# Autodesk Inventor assembly: puertas
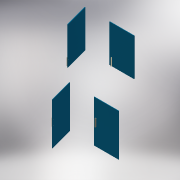
[picture p0: Inventor's stored thumbnail of the model, 180x180]
Saved by Autodesk Inventor 2016 (Build 200138000, 138)
## iProperties
Created: 2015-11-25
Part Number: puertas
Document SubType Name: Assembly
Designer: Daniela
Author: Daniela
## Documents named in this file (4)
- C:\Users\Sebastian\Desktop\sebas\trabajos\COCINA FINAAAAAAAAAAAL\COCINA FINAAAAAAAAAAAL\Cocina\Cocina\puertas.iam
- C:\Users\Sebastian\Desktop\sebas\trabajos\COCINA FINAAAAAAAAAAAL\COCINA FINAAAAAAAAAAAL\Cocina\Cocina\manija.ipt
- C:\Users\Sebastian\Desktop\sebas\trabajos\COCINA FINAAAAAAAAAAAL\COCINA FINAAAAAAAAAAAL\Cocina\Cocina\puerta_inf.ipt
- C:\Users\Sebastian\Desktop\sebas\trabajos\COCINA FINAAAAAAAAAAAL\COCINA FINAAAAAAAAAAAL\Cocina\Cocina\puerta_sup.ipt
## Components (6 placed, 3 different names)
1. puerta_inf:1 — Coincidencia:1, Coincidencia:2, Coincidencia:3, Coincidencia:4, Coincidencia:5, Coincidencia:6, Nivelación:1, Coincidencia:7, Nivelación:2
2. manija:1 — Coincidencia:4, Coincidencia:5, Coincidencia:6
3. manija:2 — Coincidencia:1, Coincidencia:2, Coincidencia:3
4. puerta_sup:1 — Nivelación:1, Coincidencia:7, Nivelación:2, Coincidencia:8, Coincidencia:9, Coincidencia:10, Coincidencia:11, Coincidencia:12, Coincidencia:13
5. manija:3 — Coincidencia:11, Coincidencia:12, Coincidencia:13
6. manija:4 — Coincidencia:8, Coincidencia:9, Coincidencia:10
## Relationships (15: Mate 13, Flush 2)
- Coincidencia:1 [Mate]: puerta_inf:1 ↔ manija:2
- Coincidencia:2 [Mate]: puerta_inf:1 ↔ manija:2
- Coincidencia:3 [Mate]: puerta_inf:1 ↔ manija:2
- Coincidencia:4 [Mate]: puerta_inf:1 ↔ manija:1
- Coincidencia:5 [Mate]: puerta_inf:1 ↔ manija:1
- Coincidencia:6 [Mate]: puerta_inf:1 ↔ manija:1
- Nivelación:1 [Flush] (300 mm): puerta_inf:1 ↔ puerta_sup:1
- Coincidencia:7 [Mate] (390 mm): puerta_inf:1 ↔ puerta_sup:1
- Nivelación:2 [Flush]: puerta_inf:1 ↔ puerta_sup:1
- Coincidencia:8 [Mate]: puerta_sup:1 ↔ manija:4
- Coincidencia:9 [Mate]: puerta_sup:1 ↔ manija:4
- Coincidencia:10 [Mate]: puerta_sup:1 ↔ manija:4
- Coincidencia:11 [Mate]: puerta_sup:1 ↔ manija:3
- Coincidencia:12 [Mate]: puerta_sup:1 ↔ manija:3
- Coincidencia:13 [Mate]: puerta_sup:1 ↔ manija:3
